# Autodesk Inventor assembly: 組合檔
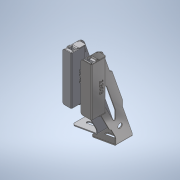
[picture p0: Inventor's stored thumbnail of the model, 180x180]
Saved by Autodesk Inventor 2020 (Build 240168000, 168)
## iProperties
Created: 2015-11-28
Part Number: 組合檔
Document SubType Name: Assembly
Designer: 設計製圖
Author: 設計製圖
## Documents named in this file (3)
- D:\資料庫\設計-3D Project\【May club 】\得利卡-車頂燈架\模型、圖面\白鐵版本(#11.02)\概念稿-資料\差異對比.iam
- D:\資料庫\設計-3D Project\【May club 】\得利卡-車頂燈架\模型、圖面\白鐵版本(#11.02)\概念稿-資料\短-車頂燈架-組合(#11.02).iam
- D:\資料庫\設計-3D Project\【May club 】\得利卡-車頂燈架\模型、圖面\車頂燈架短-組合(白鐵).iam
## Components (2 placed, 2 different names)
1. 短-車頂燈架-組合(#11.02):1 [sub-assembly] — 齊平:1, 齊平:2, 齊平:3
2. 車頂燈架短-組合(白鐵):1 [sub-assembly] — 齊平:1, 齊平:2, 齊平:3
## Relationships (3: Flush 3)
- 齊平:1 [Flush]: 短-車頂燈架-組合(#11.02):1 ↔ 車頂燈架短-組合(白鐵):1
- 齊平:2 [Flush]: 短-車頂燈架-組合(#11.02):1 ↔ 車頂燈架短-組合(白鐵):1
- 齊平:3 [Flush]: 短-車頂燈架-組合(#11.02):1 ↔ 車頂燈架短-組合(白鐵):1
